# Autodesk Inventor assembly: HF-Kabelführung-Top-Assembly
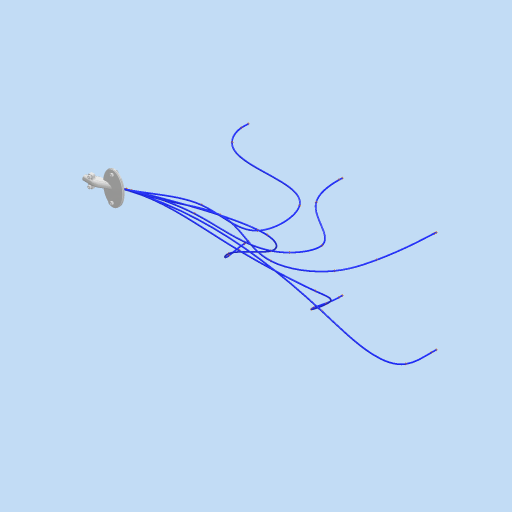
[picture p0: Inventor's stored thumbnail of the model, 512x512]
Saved by Autodesk Inventor 2023.2 (Build 272271000, 271)
## iProperties
Created: 2024-02-09
Part Number: HF-Kabelführung-Top-Assembly
Document SubType Name: Assembly
Designer: Nils Bade
Author: Nils Bade
## Documents named in this file (7)
- C:\Users\nilsb\Documents\Inventor\Projektarbeit-Bade\RatRig_Bade\HF-Kabelführung Measurement Chamber\HF-Kabelführung-Top-Assembly.iam
- C:\Users\nilsb\Documents\Inventor\Projektarbeit-Bade\RatRig_Bade\HF-Kabelführung Measurement Chamber\HF-Kabeldurchführung-TopPanel-Base.ipt
- C:\Users\nilsb\Documents\Inventor\Projektarbeit-Bade\RatRig_Bade\HF-Kabelführung Measurement Chamber\HF-Kabeldurchführung-TopPanel-Deckel.ipt
- C:\Users\nilsb\Documents\Inventor\Projektarbeit-Bade\RatRig_Bade\HF-Kabelführung Measurement Chamber\HF-Kabelführung-V2-XGantry-Kabellängen.iam
- C:\Users\nilsb\Documents\Inventor\Projektarbeit-Bade\Schrauben\Cap Head Screw M4x8 - DIN912.ipt
- C:\Users\nilsb\Documents\Inventor\Projektarbeit-Bade\RatRig_Standards\Hex Nut - M4 DIN934.ipt
- C:\Users\nilsb\Documents\Inventor\Projektarbeit-Bade\Schrauben\Cap Head Screw M4x12 - DIN912.ipt
## Components (11 placed, 6 different names)
1. HF-Kabeldurchführung-TopPanel-Base:1 — Passend:1, Passend:2, Passend:3, Passend:5, Winkel:1, Symmetrie:1, Passend:8, Winkel:5, Winkel:6, Passend:20, Passend:21, Passend:24, Passend:25
2. HF-Kabeldurchführung-TopPanel-Deckel:1 — Passend:1, Passend:2, Passend:3, Symmetrie:1, Passend:14, Passend:15, Passend:16, Passend:17
3. HF-Kabelführung-V2-XGantry-Kabellängen:1 [sub-assembly] — Winkel:2, Winkel:3, Winkel:4, Passend:9
4. Cap Head Screw M4x8 - DIN912:1 — Passend:14, Passend:17, Passend:19
5. Cap Head Screw M4x8 - DIN912:2 — Passend:15, Passend:16, Passend:18
6. Cap Head Screw M4x12 - DIN912:1
7. Cap Head Screw M4x12 - DIN912:2
8. Hex Nut - M4 DIN934:1 — Passend:19, Winkel:6, Passend:21
9. Hex Nut - M4 DIN934:2 — Passend:18, Winkel:5, Passend:20
10. Hex Nut - M4 DIN934:3 — Passend:24
11. Hex Nut - M4 DIN934:4 — Passend:25
## Relationships (31: Mate 24, Angle 6, Symmetry 1)
- Passend:1 [Mate]: HF-Kabeldurchführung-TopPanel-Base:1 ↔ HF-Kabeldurchführung-TopPanel-Deckel:1
- Passend:2 [Mate]: HF-Kabeldurchführung-TopPanel-Base:1 ↔ HF-Kabeldurchführung-TopPanel-Deckel:1
- Passend:3 [Mate]: HF-Kabeldurchführung-TopPanel-Base:1 ↔ HF-Kabeldurchführung-TopPanel-Deckel:1
- Passend:5 [Mate]: HF-Kabeldurchführung-TopPanel-Base:1
- Winkel:1 [Angle] (90 deg): HF-Kabeldurchführung-TopPanel-Base:1
- Symmetrie:1: HF-Kabeldurchführung-TopPanel-Base:1 ↔ HF-Kabeldurchführung-TopPanel-Deckel:1
- Passend:6 [Mate]
- Passend:7 [Mate]
- Passend:8 [Mate]: HF-Kabeldurchführung-TopPanel-Base:1
- Winkel:2 [Angle] (180 deg): HF-Kabelführung-V2-XGantry-Kabellängen:1
- Winkel:3 [Angle] (0 deg): HF-Kabelführung-V2-XGantry-Kabellängen:1
- Winkel:4 [Angle] (180 deg): HF-Kabelführung-V2-XGantry-Kabellängen:1
- Passend:9 [Mate]: HF-Kabelführung-V2-XGantry-Kabellängen:1
- [Mate]: HF-Kabeldurchführung-TopPanel-Deckel:1 ↔ Cap Head Screw M4x12 - DIN912:1
- [Mate]: HF-Kabeldurchführung-TopPanel-Deckel:1 ↔ Cap Head Screw M4x12 - DIN912:2
- [Mate]: HF-Kabeldurchführung-TopPanel-Deckel:1 ↔ Cap Head Screw M4x12 - DIN912:2
- [Mate]: HF-Kabeldurchführung-TopPanel-Deckel:1 ↔ Cap Head Screw M4x12 - DIN912:1
- Passend:14 [Mate]: HF-Kabeldurchführung-TopPanel-Deckel:1 ↔ Cap Head Screw M4x8 - DIN912:1
- Passend:15 [Mate]: HF-Kabeldurchführung-TopPanel-Deckel:1 ↔ Cap Head Screw M4x8 - DIN912:2
- Passend:16 [Mate]: HF-Kabeldurchführung-TopPanel-Deckel:1 ↔ Cap Head Screw M4x8 - DIN912:2
- Passend:17 [Mate]: HF-Kabeldurchführung-TopPanel-Deckel:1 ↔ Cap Head Screw M4x8 - DIN912:1
- Passend:18 [Mate]: Cap Head Screw M4x8 - DIN912:2 ↔ Hex Nut - M4 DIN934:2
- Passend:19 [Mate]: Cap Head Screw M4x8 - DIN912:1 ↔ Hex Nut - M4 DIN934:1
- Winkel:5 [Angle] (0 deg): HF-Kabeldurchführung-TopPanel-Base:1 ↔ Hex Nut - M4 DIN934:2
- Winkel:6 [Angle] (0 deg): HF-Kabeldurchführung-TopPanel-Base:1 ↔ Hex Nut - M4 DIN934:1
- Passend:20 [Mate]: HF-Kabeldurchführung-TopPanel-Base:1 ↔ Hex Nut - M4 DIN934:2
- Passend:21 [Mate]: HF-Kabeldurchführung-TopPanel-Base:1 ↔ Hex Nut - M4 DIN934:1
- [Mate]: Cap Head Screw M4x12 - DIN912:2 ↔ Hex Nut - M4 DIN934:3
- [Mate]: Cap Head Screw M4x12 - DIN912:1 ↔ Hex Nut - M4 DIN934:4
- Passend:24 [Mate] (3 mm): HF-Kabeldurchführung-TopPanel-Base:1 ↔ Hex Nut - M4 DIN934:3
- Passend:25 [Mate] (3 mm): HF-Kabeldurchführung-TopPanel-Base:1 ↔ Hex Nut - M4 DIN934:4
